# Autodesk Inventor assembly: Carriage_Assembly
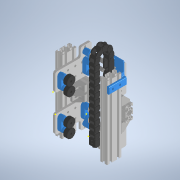
[picture p0: Inventor's stored thumbnail of the model, 180x180]
Saved by Autodesk Inventor 2021 (Build 250183000, 183)
## iProperties
Created: 2021-09-08
Part Number: Carriage_Assembly
Document SubType Name: Assembly
Designer: Jorian Brusind
Author: Jorian Brusind
## Documents named in this file (12)
- C:\Users\Jorian Brusind\Documents\GitHub\PersonalProjects\HyperRail\Inventor Files\Carriage_Assembly.iam
- C:\Users\Jorian Brusind\Documents\GitHub\PersonalProjects\Inventor Projects\Useful models\8020_Sets\IPT_20_Series\IPT_20_Series\20-2040_200mm.ipt
- C:\Users\Jorian Brusind\Documents\GitHub\PersonalProjects\Inventor Projects\Useful models\8020_Sets\IPT_20_Series\IPT_20_Series\20-2040_150mm.ipt
- C:\Users\Jorian Brusind\Documents\GitHub\PersonalProjects\HyperRail\Inventor Files\X_CarriageL_V2_0_Short.iam
- C:\Users\Jorian Brusind\Documents\GitHub\PersonalProjects\HyperRail\Inventor Files\X_CarriageR_V2_0_Short.iam
- C:\Users\Jorian Brusind\Documents\GitHub\PersonalProjects\HyperRail\Inventor Files\X_CarriageR_V2_0.iam
- C:\Users\Jorian Brusind\Documents\GitHub\PersonalProjects\HyperRail\Inventor Files\X_Carriage_V2_0.iam
- C:\Users\Jorian Brusind\Documents\GitHub\PersonalProjects\HyperRail\Inventor Files\Cable_Guide_End.ipt
- C:\Users\Jorian Brusind\Documents\GitHub\PersonalProjects\HyperRail\Inventor Files\17mmBeltGuide.ipt
- C:\Users\Jorian Brusind\Documents\GitHub\PersonalProjects\Inventor Projects\Useful models\8020_Sets\IPT_20_Series\Extra_20_Series\8020_14056m\14056_m.ipt
- C:\Users\Jorian Brusind\Documents\GitHub\PersonalProjects\Inventor Projects\Useful models\Metric Spacer_Standoffs\hex spacer standoff nut M5 L20.ipt
- C:\Users\Jorian Brusind\Documents\GitHub\PersonalProjects\HyperRail\Inventor Files\3mm_Spacer.ipt
## Components (23 placed, 11 different names)
1. 20-2040_200mm:1 — Mate:1, Flush:1, Mate:2, Flush:2, Mate:3, Mate:4, Mate:5, Mate:6, Mate:7, Flush:3, Mate:9, Flush:6, Flush:7, Flush:11, Flush:12, Mate:24, Mate:25, Mate:29
2. 20-2040_200mm:2 — Mate:10, Mate:11, Flush:5, Mate:12, Mate:13, Flush:6, Flush:7, Mate:15, Flush:8, Mate:16, Mate:17, Mate:18, Mate:19, Flush:9, Flush:10
3. 20-2040_150mm:1 — Flush:3, Mate:8, Mate:9, Mate:20, Mate:21, Mate:22, Mate:23, Mate:26, Flush:14, Mate:27, Flush:15
4. X_CarriageL_V2_0_Short:1 [sub-assembly] — Mate:10, Flush:5, Mate:13, Mate:45, Mate:48
5. X_CarriageR_V2_0_Short:1 [sub-assembly] — Mate:11, Mate:12, Mate:30, Mate:42, Mate:44, Mate:46, Mate:47
6. X_CarriageR_V2_0:1 [sub-assembly] — Mate:1, Flush:1, Mate:2, Mate:8, Mate:32, Mate:33, Mate:34, Mate:39, Mate:40
7. X_Carriage_V2_0:1 [sub-assembly] — Flush:2, Mate:3, Mate:4, Mate:35, Mate:37, Mate:38, Mate:41, Mate:43
8. Cable_Guide_End:1 — Mate:15, Flush:8, Mate:16
9. 17mmBeltGuide:1 — Mate:17, Mate:30
10. 14056_m:1 — Mate:19, Mate:21, Flush:9
11. 14056_m:2 — Mate:18, Mate:20, Flush:10
12. 14056_m:3 — Mate:22, Flush:12, Flush:13
13. 14056_m:4 — Mate:23, Flush:11, Flush:13, Mate:24
14. 14056_m:5 — Mate:27, Mate:29, Flush:15
15. 14056_m:6 — Mate:25, Mate:26, Flush:14
16. hex spacer standoff nut M5 L20:1 — Mate:32, Flush:17, Mate:39
17. hex spacer standoff nut M5 L20:2 — Mate:35, Mate:41
18. hex spacer standoff nut M5 L20:3 — Mate:34, Mate:40
19. hex spacer standoff nut M5 L20:4 — Mate:33, Flush:17, Mate:49, Mate:50
20. hex spacer standoff nut M5 L20:5 — Mate:37, Flush:16, Mate:38, Mate:42
21. hex spacer standoff nut M5 L20:6 — Flush:16, Mate:43, Mate:44
22. 3mm_Spacer:1 — Mate:46, Mate:47
23. 3mm_Spacer:2 — Mate:45, Mate:48, Mate:49, Mate:50
## Relationships (62: Mate 46, Flush 16)
- Mate:1: 20-2040_200mm:1 ↔ X_CarriageR_V2_0:1
- Flush:1: 20-2040_200mm:1 ↔ X_CarriageR_V2_0:1
- Mate:2 (5 mm): 20-2040_200mm:1 ↔ X_CarriageR_V2_0:1
- Flush:2: 20-2040_200mm:1 ↔ X_Carriage_V2_0:1
- Mate:3: 20-2040_200mm:1 ↔ X_Carriage_V2_0:1
- Mate:4 (5 mm): 20-2040_200mm:1 ↔ X_Carriage_V2_0:1
- Mate:5: 20-2040_200mm:1
- Mate:6: 20-2040_200mm:1
- Mate:7: 20-2040_200mm:1
- Flush:3: 20-2040_200mm:1 ↔ 20-2040_150mm:1
- Mate:8 (5 mm): 20-2040_150mm:1 ↔ X_CarriageR_V2_0:1
- Mate:9 (5 mm): 20-2040_200mm:1 ↔ 20-2040_150mm:1
- Mate:10: 20-2040_200mm:2 ↔ X_CarriageL_V2_0_Short:1
- Mate:11: 20-2040_200mm:2 ↔ X_CarriageR_V2_0_Short:1
- Flush:5: 20-2040_200mm:2 ↔ X_CarriageL_V2_0_Short:1
- Mate:12 (3 mm): 20-2040_200mm:2 ↔ X_CarriageR_V2_0_Short:1
- Mate:13 (3 mm): 20-2040_200mm:2 ↔ X_CarriageL_V2_0_Short:1
- Flush:6: 20-2040_200mm:1 ↔ 20-2040_200mm:2
- Flush:7: 20-2040_200mm:1 ↔ 20-2040_200mm:2
- Mate:15: 20-2040_200mm:2 ↔ Cable_Guide_End:1
- Flush:8: 20-2040_200mm:2 ↔ Cable_Guide_End:1
- Mate:16: 20-2040_200mm:2 ↔ Cable_Guide_End:1
- Mate:17: 20-2040_200mm:2 ↔ 17mmBeltGuide:1
- Mate:18: 20-2040_200mm:2 ↔ 14056_m:2
- Mate:19: 20-2040_200mm:2 ↔ 14056_m:1
- Mate:20: 20-2040_150mm:1 ↔ 14056_m:2
- Mate:21: 20-2040_150mm:1 ↔ 14056_m:1
- Flush:9: 20-2040_200mm:2 ↔ 14056_m:1
- Flush:10: 20-2040_200mm:2 ↔ 14056_m:2
- Mate:22: 20-2040_150mm:1 ↔ 14056_m:3
- Mate:23: 20-2040_150mm:1 ↔ 14056_m:4
- Flush:11: 20-2040_200mm:1 ↔ 14056_m:4
- Flush:12: 20-2040_200mm:1 ↔ 14056_m:3
- Flush:13: 14056_m:3 ↔ 14056_m:4
- Mate:24: 20-2040_200mm:1 ↔ 14056_m:4
- Mate:25: 20-2040_200mm:1 ↔ 14056_m:6
- Mate:26: 20-2040_150mm:1 ↔ 14056_m:6
- Flush:14: 20-2040_150mm:1 ↔ 14056_m:6
- Mate:27: 20-2040_150mm:1 ↔ 14056_m:5
- Mate:29: 20-2040_200mm:1 ↔ 14056_m:5
- Flush:15: 20-2040_150mm:1 ↔ 14056_m:5
- Mate:30: X_CarriageR_V2_0_Short:1 ↔ 17mmBeltGuide:1
- Mate:32: X_CarriageR_V2_0:1 ↔ hex spacer standoff nut M5 L20:1
- Mate:33: X_CarriageR_V2_0:1 ↔ hex spacer standoff nut M5 L20:4
- Mate:34: X_CarriageR_V2_0:1 ↔ hex spacer standoff nut M5 L20:3
- Mate:35: X_Carriage_V2_0:1 ↔ hex spacer standoff nut M5 L20:2
- Mate:37: X_Carriage_V2_0:1 ↔ hex spacer standoff nut M5 L20:5
- Flush:16: hex spacer standoff nut M5 L20:5 ↔ hex spacer standoff nut M5 L20:6
- Mate:38: X_Carriage_V2_0:1 ↔ hex spacer standoff nut M5 L20:5
- Flush:17: hex spacer standoff nut M5 L20:1 ↔ hex spacer standoff nut M5 L20:4
- Mate:39: X_CarriageR_V2_0:1 ↔ hex spacer standoff nut M5 L20:1
- Mate:40: X_CarriageR_V2_0:1 ↔ hex spacer standoff nut M5 L20:3
- Mate:41: X_Carriage_V2_0:1 ↔ hex spacer standoff nut M5 L20:2
- Mate:42: X_CarriageR_V2_0_Short:1 ↔ hex spacer standoff nut M5 L20:5
- Mate:43: X_Carriage_V2_0:1 ↔ hex spacer standoff nut M5 L20:6
- Mate:44: X_CarriageR_V2_0_Short:1 ↔ hex spacer standoff nut M5 L20:6
- Mate:45: X_CarriageL_V2_0_Short:1 ↔ 3mm_Spacer:2
- Mate:46 (3 mm): X_CarriageR_V2_0_Short:1 ↔ 3mm_Spacer:1
- Mate:47: X_CarriageR_V2_0_Short:1 ↔ 3mm_Spacer:1
- Mate:48 (3 mm): X_CarriageL_V2_0_Short:1 ↔ 3mm_Spacer:2
- Mate:49: hex spacer standoff nut M5 L20:4 ↔ 3mm_Spacer:2
- Mate:50: hex spacer standoff nut M5 L20:4 ↔ 3mm_Spacer:2
